# Autodesk Inventor assembly: Assembly5
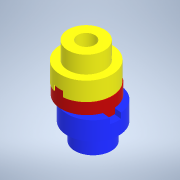
[picture p0: Inventor's stored thumbnail of the model, 180x180]
Saved by Autodesk Inventor 2020 (Build 240168000, 168)
## iProperties
Created: 2021-04-23
Part Number: Assembly5
Document SubType Name: Assembly
Designer: Sameer
Author: Sameer
## Documents named in this file (3)
- J:\Saad Khan\Study\Degree\4 Semester\Kinetics of Machinery\MP\Oldham Coupling - KoM MP.iam
- J:\Saad Khan\Study\Degree\4 Semester\Kinetics of Machinery\MP\M2020002 - Piyush Dhatrak.ipt
- J:\Saad Khan\Study\Degree\4 Semester\Kinetics of Machinery\MP\M2020001 - Khan Saad.ipt
## Components (3 placed, 2 different names)
1. M2020002 - Piyush Dhatrak:1 — Mate:1, Flush:1, Mate:2, Mate:3, Angle:1
2. M2020001 - Khan Saad:1 — Mate:2, Mate:3, Mate:4, Mate:5
3. M2020002 - Piyush Dhatrak:2 — Mate:4, Mate:5, Mate:6, Mate:7
## Relationships (9: Mate 7, Flush 1, Angle 1)
- Mate:1: M2020002 - Piyush Dhatrak:1
- Flush:1: M2020002 - Piyush Dhatrak:1
- Mate:2 (2 mm): M2020002 - Piyush Dhatrak:1 ↔ M2020001 - Khan Saad:1
- Mate:3: M2020002 - Piyush Dhatrak:1 ↔ M2020001 - Khan Saad:1
- Mate:4 (2 mm): M2020001 - Khan Saad:1 ↔ M2020002 - Piyush Dhatrak:2
- Mate:5: M2020001 - Khan Saad:1 ↔ M2020002 - Piyush Dhatrak:2
- Mate:6: M2020002 - Piyush Dhatrak:2
- Mate:7 (20 mm): M2020002 - Piyush Dhatrak:2
- Angle:1 (186 deg): M2020002 - Piyush Dhatrak:1
